# Autodesk Inventor assembly: Hobbyhh D3530 910KV
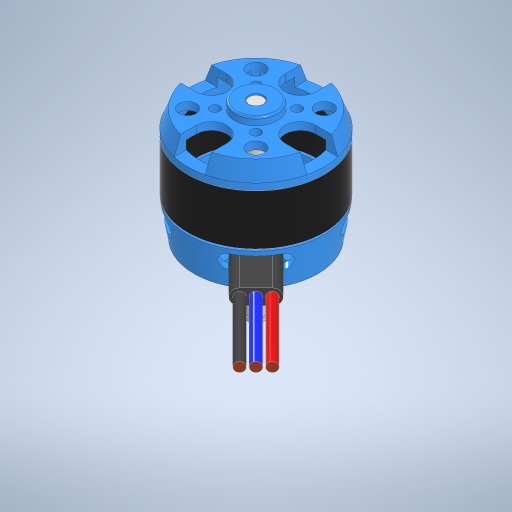
[picture p0: Inventor's stored thumbnail of the model, 512x512]
Saved by Autodesk Inventor 2023.2 (Build 272271000, 271)
## iProperties
Created: 2022-07-28
Part Number: Hobbyhh D3530 910KV
Document SubType Name: Assembly
Designer: Nathan Cai
Mass: 90 g
Surface Area: 112.738 cm^2
Volume: 9.51348 cm^3
Density: 9.46026 g/cm^3
Author: Nathan Cai
## Documents named in this file (4)
- C:\Users\Nathan Cai\Documents\Inventor\Moon Cake V0.16\Hobbyhh D3530 910KV\Hobbyhh D3530 910KV.iam
- C:\Users\Nathan Cai\Documents\Inventor\Moon Cake V0.16\Hobbyhh D3530 910KV\BASE.iam
- C:\Users\Nathan Cai\Documents\Inventor\Moon Cake V0.16\Hobbyhh D3530 910KV\CAN.iam
- C:\Users\Nathan Cai\Documents\Inventor\Moon Cake V0.16\Hobbyhh D3530 910KV\BEARING.ipt
## Components (3 placed, 3 different names)
1. BASE:1 [sub-assembly] — Mate:1, Mate:2, Mate:3
2. CAN:1 [sub-assembly] — Mate:1, Mate:2, Mate:4
3. BEARING:1 — Mate:3, Mate:4
## Relationships (4: Mate 4)
- Mate:1: BASE:1 ↔ CAN:1
- Mate:2 (-29 mm): BASE:1 ↔ CAN:1
- Mate:3: BASE:1 ↔ BEARING:1
- Mate:4: CAN:1 ↔ BEARING:1
